# Autodesk Inventor assembly: Сборка штурвал
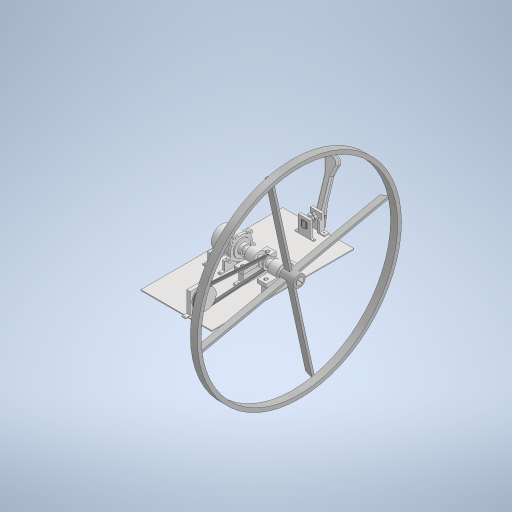
[picture p0: Inventor's stored thumbnail of the model, 512x512]
Saved by Autodesk Inventor 2023 (Build 270158000, 158)
## iProperties
Created: 2022-05-01
Part Number: Сборка штурвал
Document SubType Name: Assembly
Designer: User
Author: User
## Documents named in this file (19)
- D:\Стойка\VR-simulator-3D-models\Механизм\Сборка штурвал.iam
- D:\Стойка\VR-simulator-3D-models\Механизм\Маховик.ipt
- D:\Стойка\VR-simulator-3D-models\Механизм\Вал.ipt
- D:\Стойка\VR-simulator-3D-models\Механизм\Диск (маховик, вал).ipt
- D:\Стойка\VR-simulator-3D-models\Механизм\Стена 16 мм отверстие.ipt
- D:\Стойка\VR-simulator-3D-models\Механизм\Механизм.ipt
- D:\Стойка\VR-simulator-3D-models\Механизм\Подшипник с лапками.ipt
- D:\Стойка\VR-simulator-3D-models\Механизм ручки\Сборка ручка.iam
- D:\Стойка\VR-simulator-3D-models\Механизм\Шкив большой.ipt
- D:\Стойка\VR-simulator-3D-models\Механизм\Подставка подшипника.ipt
- D:\Стойка\VR-simulator-3D-models\Механизм\Шкив малый.ipt
- D:\Стойка\VR-simulator-3D-models\Механизм\Part38.ipt
- D:\Стойка\VR-simulator-3D-models\Механизм\Штурвал.ipt
- D:\Стойка\VR-simulator-3D-models\Механизм\Болт маховика.ipt
- D:\Стойка\VR-simulator-3D-models\Механизм\Двигатель.ipt
- D:\Стойка\VR-simulator-3D-models\Механизм\Сборка штурвал\Мастер проектирования\Передача клиновым ремнем4.iam
- D:\Стойка\VR-simulator-3D-models\Механизм\Муфта штурвал, двигатель.ipt
- D:\Стойка\VR-simulator-3D-models\Механизм\Мотор стенка.ipt
- D:\Стойка\VR-simulator-3D-models\Механизм\Стенка энкодера штурвала.ipt
## Components (22 placed, 18 different names)
1. Стена 16 мм отверстие:1 — Заподлицо:1
2. Стена 16 мм отверстие:2 — Заподлицо:1
3. Механизм:1 — Совмещение:18, Заподлицо:2, Совмещение:31, Совмещение:32, Заподлицо:7, Совмещение:40, Совмещение:42, Совмещение:80, Совмещение:81, Совмещение:85
4. Подшипник с лапками:1 — Цилиндрический:22, Заподлицо:6, Заподлицо:10, Совмещение:88
5. Подшипник с лапками:2 — Цилиндрический:22, Совмещение:21, Заподлицо:3, Совмещение:75, Заподлицо:9, Совмещение:77
6. Сборка ручка:1 [sub-assembly] — Совмещение:18, Заподлицо:2, Совмещение:42
7. Вал:1 — Совмещение:21, Совмещение:22, Совмещение:23, Совмещение:24, Совмещение:59, Совмещение:72, Совмещение:73, Совмещение:76
8. Диск (маховик, вал):1 — Совмещение:22, Совмещение:23, Совмещение:24, Совмещение:27, С поворотом:2, Совмещение:77
9. Маховик:1 — Совмещение:27, Совмещение:56, Совмещение:57, С поворотом:2
10. Подставка подшипника:1 — Совмещение:31, Заподлицо:6, Заподлицо:10
11. Подставка подшипника:2 — Совмещение:32, Заподлицо:3, Заподлицо:7, Совмещение:40, Совмещение:75, Заподлицо:9
12. Шкив малый:1 — Совмещение:59, Совмещение:68, Заподлицо:8, Совмещение:69, Совмещение:76
13. Штурвал:1 — Совмещение:54, Совмещение:55, Совмещение:56, Совмещение:57
14. Болт маховика:1 — Совмещение:54, Совмещение:55
15. Двигатель:1 — Совмещение:70, Совмещение:71, Совмещение:73, Совмещение:78, Совмещение:79, Совмещение:82, Совмещение:83, Заподлицо:11
16. Шкив большой:2 — Совмещение:63, Совмещение:64, Совмещение:66, Заподлицо:8, Совмещение:87
17. Part38:2 — Совмещение:63, Совмещение:64, Совмещение:86
18. Передача клиновым ремнем:1 [sub-assembly] — Совмещение:66, Совмещение:68, Совмещение:69
19. Муфта штурвал, двигатель:1 — Совмещение:70, Совмещение:71, Совмещение:72, Совмещение:88
20. Мотор стенка:1 — Совмещение:79, Совмещение:81, Совмещение:82, Совмещение:83
21. Мотор стенка:2 — Совмещение:78, Совмещение:80, Заподлицо:11
22. Стенка энкодера штурвала:1 — Совмещение:85, Совмещение:86, Совмещение:87
## Relationships (48: Mate 37, Flush 9, CylindricalJoint 1, RevoluteJoint 1)
- Заподлицо:1 [Flush]: Стена 16 мм отверстие:1 ↔ Стена 16 мм отверстие:2
- Совмещение:18 [Mate]: Механизм:1 ↔ Сборка ручка:1
- Заподлицо:2 [Flush]: Механизм:1 ↔ Сборка ручка:1
- Цилиндрический:22 [CylindricalJoint]: Подшипник с лапками:1 ↔ Подшипник с лапками:2
- Совмещение:21 [Mate]: Подшипник с лапками:2 ↔ Вал:1
- Совмещение:22 [Mate]: Вал:1 ↔ Диск (маховик, вал):1
- Совмещение:23 [Mate]: Вал:1 ↔ Диск (маховик, вал):1
- Совмещение:24 [Mate]: Вал:1 ↔ Диск (маховик, вал):1
- Совмещение:27 [Mate]: Диск (маховик, вал):1 ↔ Маховик:1
- Совмещение:31 [Mate]: Механизм:1 ↔ Подставка подшипника:1
- Совмещение:32 [Mate]: Механизм:1 ↔ Подставка подшипника:2
- Заподлицо:3 [Flush]: Подшипник с лапками:2 ↔ Подставка подшипника:2
- Заподлицо:6 [Flush]: Подшипник с лапками:1 ↔ Подставка подшипника:1
- Заподлицо:7 [Flush]: Механизм:1 ↔ Подставка подшипника:2
- Совмещение:40 [Mate]: Механизм:1 ↔ Подставка подшипника:2
- Совмещение:42 [Mate]: Механизм:1 ↔ Сборка ручка:1
- Совмещение:54 [Mate]: Штурвал:1 ↔ Болт маховика:1
- Совмещение:55 [Mate]: Штурвал:1 ↔ Болт маховика:1
- Совмещение:56 [Mate]: Маховик:1 ↔ Штурвал:1
- Совмещение:57 [Mate]: Маховик:1 ↔ Штурвал:1
- С поворотом:2 [RevoluteJoint]: Диск (маховик, вал):1 ↔ Маховик:1
- Совмещение:59 [Mate]: Вал:1 ↔ Шкив малый:1
- Совмещение:63 [Mate]: Шкив большой:2 ↔ Part38:2
- Совмещение:64 [Mate]: Шкив большой:2 ↔ Part38:2
- Совмещение:66 [Mate]: Шкив большой:2 ↔ Передача клиновым ремнем:1
- Совмещение:68 [Mate]: Шкив малый:1 ↔ Передача клиновым ремнем:1
- Заподлицо:8 [Flush]: Шкив малый:1 ↔ Шкив большой:2
- Совмещение:69 [Mate]: Шкив малый:1 ↔ Передача клиновым ремнем:1
- Совмещение:70 [Mate]: Двигатель:1 ↔ Муфта штурвал, двигатель:1
- Совмещение:71 [Mate]: Двигатель:1 ↔ Муфта штурвал, двигатель:1
- Совмещение:72 [Mate]: Вал:1 ↔ Муфта штурвал, двигатель:1
- Совмещение:73 [Mate]: Вал:1 ↔ Двигатель:1
- Совмещение:75 [Mate]: Подшипник с лапками:2 ↔ Подставка подшипника:2
- Заподлицо:9 [Flush]: Подшипник с лапками:2 ↔ Подставка подшипника:2
- Заподлицо:10 [Flush]: Подшипник с лапками:1 ↔ Подставка подшипника:1
- Совмещение:76 [Mate]: Вал:1 ↔ Шкив малый:1
- Совмещение:77 [Mate]: Подшипник с лапками:2 ↔ Диск (маховик, вал):1
- Совмещение:78 [Mate]: Двигатель:1 ↔ Мотор стенка:2
- Совмещение:79 [Mate]: Двигатель:1 ↔ Мотор стенка:1
- Совмещение:80 [Mate]: Механизм:1 ↔ Мотор стенка:2
- Совмещение:81 [Mate]: Механизм:1 ↔ Мотор стенка:1
- Совмещение:82 [Mate]: Двигатель:1 ↔ Мотор стенка:1
- Совмещение:83 [Mate]: Двигатель:1 ↔ Мотор стенка:1
- Заподлицо:11 [Flush]: Двигатель:1 ↔ Мотор стенка:2
- Совмещение:85 [Mate]: Механизм:1 ↔ Стенка энкодера штурвала:1
- Совмещение:86 [Mate]: Part38:2 ↔ Стенка энкодера штурвала:1
- Совмещение:87 [Mate]: Шкив большой:2 ↔ Стенка энкодера штурвала:1
- Совмещение:88 [Mate]: Подшипник с лапками:1 ↔ Муфта штурвал, двигатель:1
